# Autodesk Inventor assembly: KB33-046-003 - Уголок с креплением мотора
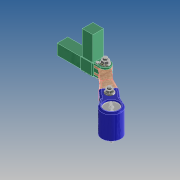
[picture p0: Inventor's stored thumbnail of the model, 180x180]
Saved by Autodesk Inventor 2020 (Build 240168000, 168)
## iProperties
Created: 2021-06-20
Part Number: KB33-046-003 - Уголок с креплением мотора
Document SubType Name: Assembly
Designer: Петров Иван
Mass: 515.916 g
Surface Area: 940.882 cm^2
Volume: 385.289 cm^3
Density: 1.33904 g/cm^3
Author: Петров Иван
## Documents named in this file (9)
- E:\IVAN\Ivan_desktop\Kvantorium\Projects\RoboPatrol\design\KB33-046-003 - Уголок с креплением мотора.iam
- E:\IVAN\Ivan_desktop\Kvantorium\Projects\RoboPatrol\design\KB33-046-003-001 - Уголок.ipt
- E:\IVAN\Ivan_desktop\Kvantorium\Projects\RoboPatrol\design\KB33-046-003-002 - Рычаг.ipt
- E:\IVAN\Ivan_desktop\Kvantorium\Projects\RoboPatrol\design\KB33-046-003-003 - Крепление.ipt
- E:\IVAN\Ivan_desktop\Kvantorium\Projects\RoboPatrol\design\standart_components\dc_gear_motor_12V_500rpm\dc_gear_motor_12V_500rpm2.ipt
- C:\Users\Петров Иван\Documents\Inventor\Content Center Files\R2020\ru-RU\GOST 7798-70\Болт M10-6gx45 ГОСТ 7798-70.ipt
- C:\Users\Петров Иван\Documents\Inventor\Content Center Files\R2020\ru-RU\ANSI B18.2.4.4M\ANSI B18.2.4.4M - M10 x 1,5.ipt
- E:\IVAN\Ivan_desktop\Kvantorium\Projects\RoboPatrol\design\KB33-046-002 - Уголок с креплением мотора\Мастер проектирования\Болтовое соединение12.iam
- C:\Users\Петров Иван\Documents\Inventor\Content Center Files\R2020\ru-RU\GOST 7798-70\Болт M10-6gx55 ГОСТ 7798-70.ipt
## Components (10 placed, 8 different names)
1. KB33-046-003-001 - Уголок:1 — Совмещение:2, Заподлицо:1, Совмещение:1, Вставка:1, Вставка:2, Совмещение:11, Совмещение:10, Совмещение:13, Совмещение:16
2. KB33-046-003-002 - Рычаг:1 — Совмещение:2, Заподлицо:1, Совмещение:1, Заподлицо:3, Совмещение:6, Совмещение:5
3. KB33-046-003-003 - Крепление:1 — Заподлицо:3, Совмещение:6, Совмещение:5, Совмещение:9, Совмещение:8, Совмещение:7, Совмещение:17, Совмещение:18, Совмещение:19
4. dc_gear_motor_12V_500rpm2:1 — Совмещение:9, Совмещение:8, Совмещение:7
5. Болт ГОСТ 7798-70 - Отозвано M10-6gx45:1 — Вставка:1
6. Гайки метрические шестигранные с фланцем - метрическая M10 x 1,5:1 — Вставка:2
7. Болтовое соединение12:1 [sub-assembly] — Совмещение:11, Совмещение:10
8. Болтовое соединение12:2 [sub-assembly] — Совмещение:13, Совмещение:16
9. Болт ГОСТ 7798-70 - Отозвано M10-6gx55:1 — Совмещение:18, Совмещение:19
10. Гайки метрические шестигранные с фланцем - метрическая M10 x 1,5:2 — Совмещение:17
## Relationships (18: Mate 13, Flush 3, Insert 2)
- Совмещение:2 [Mate]: KB33-046-003-001 - Уголок:1 ↔ KB33-046-003-002 - Рычаг:1
- Заподлицо:1 [Flush]: KB33-046-003-001 - Уголок:1 ↔ KB33-046-003-002 - Рычаг:1
- Совмещение:1 [Mate]: KB33-046-003-001 - Уголок:1 ↔ KB33-046-003-002 - Рычаг:1
- Заподлицо:3 [Flush] (-7.0385 mm): KB33-046-003-002 - Рычаг:1 ↔ KB33-046-003-003 - Крепление:1
- Совмещение:6 [Mate]: KB33-046-003-002 - Рычаг:1 ↔ KB33-046-003-003 - Крепление:1
- Совмещение:5 [Mate]: KB33-046-003-002 - Рычаг:1 ↔ KB33-046-003-003 - Крепление:1
- Совмещение:9 [Mate]: KB33-046-003-003 - Крепление:1 ↔ dc_gear_motor_12V_500rpm2:1
- Совмещение:8 [Mate]: KB33-046-003-003 - Крепление:1 ↔ dc_gear_motor_12V_500rpm2:1
- Совмещение:7 [Mate]: KB33-046-003-003 - Крепление:1 ↔ dc_gear_motor_12V_500rpm2:1
- Вставка:1 [Insert]: KB33-046-003-001 - Уголок:1 ↔ Болт ГОСТ 7798-70 - Отозвано M10-6gx45:1
- Вставка:2 [Insert]: KB33-046-003-001 - Уголок:1 ↔ Гайки метрические шестигранные с фланцем - метрическая M10 x 1,5:1
- Совмещение:11 [Mate]: KB33-046-003-001 - Уголок:1 ↔ Болтовое соединение12:1
- Совмещение:10 [Flush]: KB33-046-003-001 - Уголок:1 ↔ Болтовое соединение12:1
- Совмещение:13 [Mate]: KB33-046-003-001 - Уголок:1 ↔ Болтовое соединение12:2
- Совмещение:16 [Mate]: KB33-046-003-001 - Уголок:1 ↔ Болтовое соединение12:2
- Совмещение:17 [Mate]: KB33-046-003-003 - Крепление:1 ↔ Гайки метрические шестигранные с фланцем - метрическая M10 x 1,5:2
- Совмещение:18 [Mate]: KB33-046-003-003 - Крепление:1 ↔ Болт ГОСТ 7798-70 - Отозвано M10-6gx55:1
- Совмещение:19 [Mate]: KB33-046-003-003 - Крепление:1 ↔ Болт ГОСТ 7798-70 - Отозвано M10-6gx55:1
